# Autodesk Inventor assembly: bottom
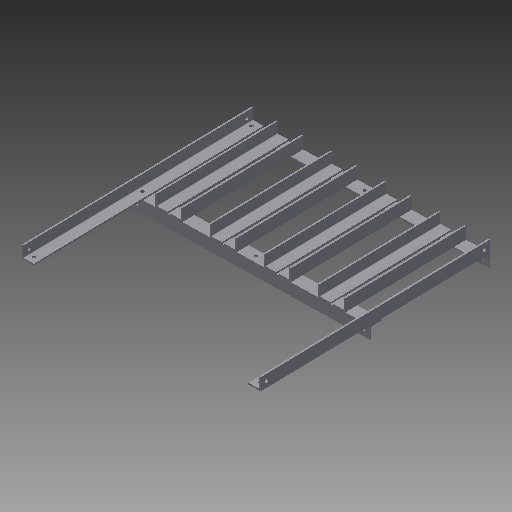
[picture p0: Inventor's stored thumbnail of the model, 512x512]
Saved by Autodesk Inventor 2017 (Build 210142000, 142)
## iProperties
Created: 2018-10-17
Part Number: bottom
Document SubType Name: Assembly
Designer: ddeboer
Author: ddeboer
## Documents named in this file (3)
- C:\Users\ddeboer\Desktop\snap_holder\top.iam
- C:\Users\ddeboer\Desktop\snap_holder\ladder.iam
- C:\Users\ddeboer\Desktop\snap_holder\channel.ipt
## Components (3 placed, 2 different names)
1. ladder:1 [sub-assembly] — Insert:3, Insert:4, Flush:1, Flush:2
2. channel:1 — Insert:3, Flush:1
3. channel:2 — Insert:4, Flush:2
## Relationships (4: Insert 2, Flush 2)
- Insert:3: ladder:1 ↔ channel:1
- Insert:4: ladder:1 ↔ channel:2
- Flush:1: ladder:1 ↔ channel:1
- Flush:2: ladder:1 ↔ channel:2
